# Autodesk Inventor assembly: Assembly
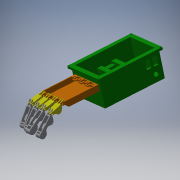
[picture p0: Inventor's stored thumbnail of the model, 180x180]
Saved by Autodesk Inventor 2019 (Build 230136000, 136)
## iProperties
Created: 2018-12-05
Part Number: Assembly
Document SubType Name: Assembly
Designer: jerem
Author: jerem
## Documents named in this file (7)
- C:\Users\jerem\Desktop\Uni Notes\MSD\Project_Hand\V1.2\Assembly.iam
- C:\Users\jerem\Desktop\Uni Notes\MSD\Project_Hand\V1.2\index.ipt
- C:\Users\jerem\Desktop\Uni Notes\MSD\Project_Hand\V1.2\finger_joins.ipt
- C:\Users\jerem\Desktop\Uni Notes\MSD\Project_Hand\V1.2\palm.ipt
- C:\Users\jerem\Desktop\Uni Notes\MSD\Project_Hand\V1.2\middle.ipt
- C:\Users\jerem\Desktop\Uni Notes\MSD\Project_Hand\V1.2\pinkie.ipt
- C:\Users\jerem\Desktop\Uni Notes\MSD\Project_Hand\V1.2\mien_arm.ipt
## Components (10 placed, 6 different names)
1. index:1 — Mate:3, Mate:4
2. finger_joins:1 — Mate:3, Mate:4, Mate:5, Mate:6
3. palm:1 — Mate:5, Mate:6, Mate:11, Mate:12, Mate:13, Mate:14, Mate:17, Mate:18, Mate:19, Mate:20, Mate:21
4. index:2
5. finger_joins:2 — Mate:13, Mate:14
6. finger_joins:3 — Mate:15, Mate:16, Mate:17, Mate:18
7. finger_joins:4 — Mate:9, Mate:10, Mate:11, Mate:12
8. middle:1 — Mate:9, Mate:10
9. pinkie:1 — Mate:15, Mate:16
10. mien_arm:1 — Mate:19, Mate:20, Mate:21
## Relationships (19: Mate 19)
- Mate:3: index:1 ↔ finger_joins:1
- Mate:4: index:1 ↔ finger_joins:1
- Mate:5: finger_joins:1 ↔ palm:1
- Mate:6: finger_joins:1 ↔ palm:1
- [Mate]: index:2 ↔ finger_joins:2
- [Mate]: index:2 ↔ finger_joins:2
- Mate:9: finger_joins:4 ↔ middle:1
- Mate:10: finger_joins:4 ↔ middle:1
- Mate:11: palm:1 ↔ finger_joins:4
- Mate:12: palm:1 ↔ finger_joins:4
- Mate:13: palm:1 ↔ finger_joins:2
- Mate:14: palm:1 ↔ finger_joins:2
- Mate:15: finger_joins:3 ↔ pinkie:1
- Mate:16: finger_joins:3 ↔ pinkie:1
- Mate:17: palm:1 ↔ finger_joins:3
- Mate:18: palm:1 ↔ finger_joins:3
- Mate:19: palm:1 ↔ mien_arm:1
- Mate:20: palm:1 ↔ mien_arm:1
- Mate:21: palm:1 ↔ mien_arm:1
## Named parameters: d10_d6 = 0 mm, d11_d7 = 0 mm
